# Autodesk Inventor assembly: assembly_gripper
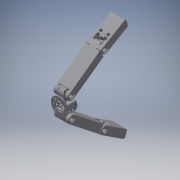
[picture p0: Inventor's stored thumbnail of the model, 180x180]
Saved by Autodesk Inventor 2018 (Build 220112000, 112)
## iProperties
Created: 2018-04-13
Part Number: assembly_gripper
Material: Genérico
Document SubType Name: Assembly
Designer: se_ma
Author: se_ma
## Documents named in this file (4)
- C:\programming\hecatonquiros\cad_models\tools\gripper\two_fingers_tensor\assembly_gripper.iam
- C:\programming\hecatonquiros\cad_models\tools\gripper\two_fingers_tensor\base.ipt
- C:\programming\hecatonquiros\cad_models\tools\gripper\two_fingers_tensor\finger_long.ipt
- C:\programming\hecatonquiros\cad_models\tools\gripper\two_fingers_tensor\finger_short.ipt
## Components (5 placed, 3 different names)
1. base:1 — Coincidencia:1, Coincidencia:2, Coincidencia:3, Coincidencia:4
2. finger_long:1 — Coincidencia:1, Coincidencia:2, Coincidencia:7, Coincidencia:8
3. finger_long:2 — Coincidencia:3, Coincidencia:4, Coincidencia:5, Coincidencia:6
4. finger_short:1 — Coincidencia:5, Coincidencia:6
5. finger_short:2 — Coincidencia:7, Coincidencia:8
## Relationships (8: Mate 8)
- Coincidencia:1 [Mate]: base:1 ↔ finger_long:1
- Coincidencia:2 [Mate]: base:1 ↔ finger_long:1
- Coincidencia:3 [Mate]: base:1 ↔ finger_long:2
- Coincidencia:4 [Mate]: base:1 ↔ finger_long:2
- Coincidencia:5 [Mate]: finger_long:2 ↔ finger_short:1
- Coincidencia:6 [Mate]: finger_long:2 ↔ finger_short:1
- Coincidencia:7 [Mate]: finger_long:1 ↔ finger_short:2
- Coincidencia:8 [Mate]: finger_long:1 ↔ finger_short:2
